# Autodesk Inventor assembly: new_assembly_auger
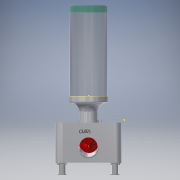
[picture p0: Inventor's stored thumbnail of the model, 180x180]
Saved by Autodesk Inventor 2019 (Build 230136000, 136)
## iProperties
Created: 2019-01-23
Part Number: new_assembly_auger
Document SubType Name: Assembly
Designer: jmc
Author: jmc
## Documents named in this file (10)
- C:\Users\l0086\Desktop\Models\CatFeeder\version4 (auger)\new_assembly_auger.iam
- C:\Users\l0086\Desktop\Models\CatFeeder\Case\version3\case_top.ipt
- C:\Users\l0086\Desktop\Models\CatFeeder\Case\version3\case_bottom.ipt
- C:\Users\l0086\Desktop\Models\CatFeeder\version4 (auger)\subassembly_jar_jarcone.iam
- C:\Users\l0086\Desktop\Models\CatFeeder\version4 (auger)\subassembly_auger_case.iam
- C:\Users\l0086\Desktop\Models\3party\Boards\ArduinoNano\arduino nano.iam
- C:\Users\l0086\Desktop\Models\3party\Boards\Raspberry Pi 3\Raspberry Pi 3.ipt
- C:\Users\l0086\Desktop\Models\3party\Trasformer\Transformer.ipt
- C:\Users\l0086\Desktop\Models\CatFeeder\Case\version2\Pata.ipt
- C:\Users\l0086\Desktop\Models\CatFeeder\Case\version2\pata_macho.ipt
## Components (15 placed, 9 different names)
1. subassembly_jar_jarcone:1 [sub-assembly] — Rigid:2
2. subassembly_auger_case:1 [sub-assembly] — Rigid:3
3. Pata:1 — Mate:6, Flush:1, Flush:2, Rotational:1
4. pata_macho:1 — Rotational:1
5. Pata:2 — Mate:8, Flush:7, Flush:8, Rotational:2
6. Pata:3 — Mate:7, Flush:3, Flush:4, Rotational:3
7. Pata:4 — Mate:9, Flush:5, Flush:6, Rotational:4
8. pata_macho:2 — Rotational:2
9. pata_macho:3 — Rotational:3
10. pata_macho:4 — Rotational:4
11. case_top:1 — Rigid:1, Rigid:2, Rigid:3
12. case_bottom:1 — Rigid:1, Mate:1, Mate:2, Mate:5, Mate:6, Flush:1, Flush:2, Mate:7, Mate:8, Mate:9, Flush:3, Flush:4, Flush:5, Flush:6, Flush:7, Flush:8
13. arduino nano:1 [sub-assembly] — Mate:5
14. Transformer:1 — Mate:1, Mate:2, Mate:4
15. Raspberry Pi 3:1 — Mate:4
## Relationships (23: Mate 8, Flush 8, RevoluteJoint 4, WeldJoint 3)
- Rigid:1 [WeldJoint]: case_top:1 ↔ case_bottom:1
- Rigid:2 [WeldJoint]: subassembly_jar_jarcone:1 ↔ case_top:1
- Rigid:3 [WeldJoint]: subassembly_auger_case:1 ↔ case_top:1
- Mate:1 (1 mm): case_bottom:1 ↔ Transformer:1
- Mate:2: case_bottom:1 ↔ Transformer:1
- Mate:4 (-2 mm): Transformer:1 ↔ Raspberry Pi 3:1
- Mate:5 (10 mm): case_bottom:1 ↔ arduino nano:1
- Mate:6: Pata:1 ↔ case_bottom:1
- Flush:1: Pata:1 ↔ case_bottom:1
- Flush:2: Pata:1 ↔ case_bottom:1
- Rotational:1 [RevoluteJoint]: Pata:1 ↔ pata_macho:1
- Mate:7: Pata:3 ↔ case_bottom:1
- Mate:8: Pata:2 ↔ case_bottom:1
- Mate:9: Pata:4 ↔ case_bottom:1
- Flush:3: Pata:3 ↔ case_bottom:1
- Flush:4: Pata:3 ↔ case_bottom:1
- Flush:5: Pata:4 ↔ case_bottom:1
- Flush:6: Pata:4 ↔ case_bottom:1
- Flush:7: Pata:2 ↔ case_bottom:1
- Flush:8: Pata:2 ↔ case_bottom:1
- Rotational:2 [RevoluteJoint]: Pata:2 ↔ pata_macho:2
- Rotational:3 [RevoluteJoint]: Pata:3 ↔ pata_macho:3
- Rotational:4 [RevoluteJoint]: Pata:4 ↔ pata_macho:4
